# Autodesk Inventor assembly: USAN_Assembly
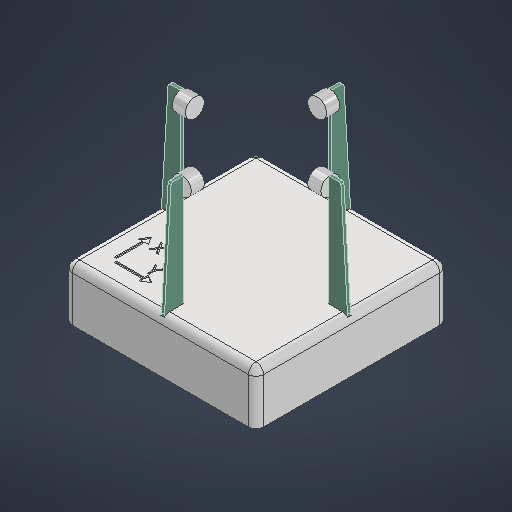
[picture p0: Inventor's stored thumbnail of the model, 512x512]
Saved by Autodesk Inventor 2025 (Build 290162010, 162A)
## iProperties
Created: 2024-10-14
Part Number: USAN_Assembly
Document SubType Name: Assembly
Designer: tzu98
Author: tzu98
## iProperties of the stored document PinSocket_1x02_P2.54mm_Vertical.iam
Created: 2024-12-02
Part Number: PinSocket_1x02_P2.54mm_Vertical
Document SubType Name: Assembly
Designer: tzu98
Author: tzu98
## iProperties of the stored document USAN_TR_r0_PCB.ipt
Created: 2024-12-02
Part Number: USAN_TR_r0_PCB
Material: Generic
Document SubType Name: Modeling
Designer: tzu98
Density: 1 g/cm^3
Appearance: Default
Mass: 1.10852 g
Surface Area: 16.7621 cm^2
Volume: 1.10852 cm^3
Author: tzu98
## iProperties of the stored document PinSocket_1x02_P254mm_Vertical.ipt
Created: 2024-12-02
Part Number: PinSocket_1x02_P254mm_Vertical
Material: Generic
Document SubType Name: Modeling
Designer: tzu98
Density: 1 g/cm^3
Appearance: Default
Mass: 0.0849448 g
Surface Area: 1.75065 cm^2
Volume: 0.0849448 cm^3
Author: tzu98
## iProperties of the stored document USAN_TR_r0.iam
Company: Kicad
Created: 2024-12-12
Part Number: USAN_TR_r0 1
Description: KiCad electronic assembly
Document SubType Name: Assembly
Designer: tzu98
Authority: Unknown
Sending System: KiCad to STEP converter
Preprocessor: Open CASCADE STEP processor 7.8
Title: USAN_TR_r0.step
Author: Pcbnew
## Documents named in this file (18)
- A:\Documente\Uni\Praxisprojekt\open-USAN\2D-US-Anemometer-Hardware\CAD\USAN_Assembly.iam
- A:\Documente\Uni\Praxisprojekt\open-USAN\2D-US-Anemometer-Hardware\CAD\Mainbody.ipt
- C:\Users\tzu98\Documents\Inventor\Content Center Files\R2025\en-US\DIN 912\DIN 912 - M3 x 0,5 x 5 x 3,75.ipt
- A:\Documente\Uni\Praxisprojekt\open-USAN\2D-US-Anemometer-Hardware\CAD\Lid.ipt
- A:\Documente\Uni\Praxisprojekt\open-USAN\2D-US-Anemometer-Hardware\CAD\Trans.ipt
- A:\Documente\Uni\Praxisprojekt\open-USAN\2D-US-Anemometer-Hardware\CAD\USAN_r0_PCB\USAN_r0_PCB.iam
- **A:\Documente\Uni\Praxisprojekt\open-USAN\2D-US-Anemometer-Hardware\CAD\USAN_Assembly.iam*LocalDocs*xAaaaqhcaAaaaaaaaAaaaqq2w3g*USAN_TR_r0.iam
- C:\Users\tzu98\Documents\Inventor\Content Center Files\R2025\en-US\DIN 7991(2)\DIN 7991 - M4x10.ipt
- A:\Documente\Uni\Praxisprojekt\open-USAN\2D-US-Anemometer-Hardware\CAD\Lid_uart.ipt
- **A:\Documente\Uni\Praxisprojekt\open-USAN\2D-US-Anemometer-Hardware\CAD\USAN_Assembly.iam*LocalDocs*xAaaaa4caAaaaaaaaAaaaqcqrCe*PinSocket_1x02_P2.54mm_Vertical.iam
- **A:\Documente\Uni\Praxisprojekt\open-USAN\2D-US-Anemometer-Hardware\CAD\USAN_Assembly.iam*LocalDocs*xAaaaagaaAaaaaaaaAaaaqncpQd*PinSocket_1x02_P254mm_Vertical.ipt
- **A:\Documente\Uni\Praxisprojekt\open-USAN\2D-US-Anemometer-Hardware\CAD\USAN_Assembly.iam*LocalDocs*xAaaaa1aaAaaaaaaaAaaaajd3Ma*USAN_TR_r0_PCB.ipt
- A:\Documente\Uni\Praxisprojekt\open-USAN\2D-US-Anemometer-Hardware\CAD\USAN_TR_r0.step
- A:\Documente\Uni\Praxisprojekt\open-USAN\2D-US-Anemometer-Hardware\CAD\USAN_Assembly\AIP\FEA\f006r4stc.fins
- A:\Documente\Uni\Praxisprojekt\open-USAN\2D-US-Anemometer-Hardware\CAD\USAN_Assembly\AIP\FEA\f006r4stc.fsat
- A:\Documente\Uni\Praxisprojekt\open-USAN\2D-US-Anemometer-Hardware\CAD\USAN_Assembly\AIP\FEA\f006r4stc.ftes
- A:\Documente\Uni\Praxisprojekt\open-USAN\2D-US-Anemometer-Hardware\CAD\USAN_Assembly\AIP\FEA\f006r4stc.fwiz
- A:\Documente\Uni\Praxisprojekt\open-USAN\2D-US-Anemometer-Hardware\CAD\USAN_Assembly\AIP\FEA\f006r4tls.fmsh
## Components (20 placed, 8 different names)
1. Mainbody:1 — Mate:4, Mate:17, Mate:18, Mate:19, Mate:26, Mate:27, Mate:28, Mate:31, Mate:32, Mate:37, Mate:38, Mate:39
2. DIN 912 - replaced by DIN EN ISO 4762 M3 x 5:1 — Insert:4
3. DIN 912 - replaced by DIN EN ISO 4762 M3 x 5:2 — Insert:3
4. DIN 912 - replaced by DIN EN ISO 4762 M3 x 5:3 — Insert:1
5. DIN 912 - replaced by DIN EN ISO 4762 M3 x 5:4 — Insert:2
6. Lid:1 — Mate:4, Mate:31, Mate:32, Mate:33, Mate:34, Mate:35, Mate:36
7. USAN_r0_PCB:1 [sub-assembly] — Mate:17, Mate:18, Mate:19, Insert:1, Insert:2, Insert:3, Insert:4
8. DIN 7991 M4x10:1 — Mate:33
9. DIN 7991 M4x10:2 — Mate:34
10. DIN 7991 M4x10:3 — Mate:35
11. DIN 7991 M4x10:4 — Mate:36
12. Lid_uart:1 — Mate:37, Mate:38, Mate:39
13. USAN_TR_r0:1 [sub-assembly] — Mate:26, Mate:27, Mate:28, Mate:29, Mate:30
14. Trans:2 — Mate:29, Mate:30
15. USAN_TR_r0:2 [sub-assembly]
16. Trans:3
17. USAN_TR_r0:3 [sub-assembly]
18. Trans:4
19. USAN_TR_r0:4 [sub-assembly]
20. Trans:5
## Component patterns: (4 elements, first: USAN_TR_r0:1 + Trans:2)
## Relationships (22: Mate 18, Insert 4)
- Mate:4: Mainbody:1 ↔ Lid:1
- Mate:17: Mainbody:1 ↔ USAN_r0_PCB:1
- Mate:18: Mainbody:1 ↔ USAN_r0_PCB:1
- Mate:19: Mainbody:1 ↔ USAN_r0_PCB:1
- Insert:1: DIN 912 - replaced by DIN EN ISO 4762 M3 x 5:3 ↔ USAN_r0_PCB:1
- Insert:2: DIN 912 - replaced by DIN EN ISO 4762 M3 x 5:4 ↔ USAN_r0_PCB:1
- Insert:3: DIN 912 - replaced by DIN EN ISO 4762 M3 x 5:2 ↔ USAN_r0_PCB:1
- Insert:4: DIN 912 - replaced by DIN EN ISO 4762 M3 x 5:1 ↔ USAN_r0_PCB:1
- Mate:26 (0.1 mm): Mainbody:1 ↔ USAN_TR_r0:1
- Mate:27: Mainbody:1 ↔ USAN_TR_r0:1
- Mate:28: Mainbody:1 ↔ USAN_TR_r0:1
- Mate:29: USAN_TR_r0:1 ↔ Trans:2
- Mate:30 (-5 mm): USAN_TR_r0:1 ↔ Trans:2
- Mate:31: Mainbody:1 ↔ Lid:1
- Mate:32: Mainbody:1 ↔ Lid:1
- Mate:33: Lid:1 ↔ DIN 7991 M4x10:1
- Mate:34: Lid:1 ↔ DIN 7991 M4x10:2
- Mate:35: Lid:1 ↔ DIN 7991 M4x10:3
- Mate:36: Lid:1 ↔ DIN 7991 M4x10:4
- Mate:37: Mainbody:1 ↔ Lid_uart:1
- Mate:38 (0.1 mm): Mainbody:1 ↔ Lid_uart:1
- Mate:39 (0.1 mm): Mainbody:1 ↔ Lid_uart:1
